# Autodesk Inventor assembly: Electrical Workbench
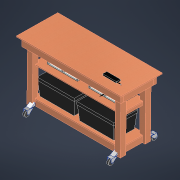
[picture p0: Inventor's stored thumbnail of the model, 180x180]
Saved by Autodesk Inventor 2022.3 (Build 263350000, 350)
## iProperties
Created: 2022-08-14
Part Number: Electrical Workbench
Document SubType Name: Assembly
Designer: hawle
Author: hawle
## Documents named in this file (25)
- G:\Robotics 2022 CAD Files\Workshop\Electrical Workbench.iam
- G:\Robotics 2022 CAD Files\Workshop\2x6x72 wood.ipt
- G:\Robotics 2022 CAD Files\Workshop\2x6x44 wood.ipt
- G:\Robotics 2022 CAD Files\Workshop\2x6x40 wood.ipt
- G:\Robotics 2022 CAD Files\Workshop\2x6x60 wood.ipt
- G:\Robotics 2022 CAD Files\Workshop\Workbench top.ipt
- G:\Robotics 2022 CAD Files\Workshop\workbench floor.ipt
- G:\Robotics 2022 CAD Files\Workshop\2x6x33 wood.ipt
- G:\Robotics 2022 CAD Files\Workshop\Workbench caster assembly.iam
- G:\Robotics 2022 CAD Files\Workshop\Power Strip.ipt
- G:\Robotics 2022 CAD Files\Game Pieces\First Tote.ipt
- G:\Robotics 2022 CAD Files\Workshop\Electrical Drawer.iam
- G:\Robotics 2022 CAD Files\Workshop\3x3x42 wood.ipt
- G:\Robotics 2022 CAD Files\Workshop\Electrical Workbench\AIP\FEA\e2dqfnm0w.fins
- G:\Robotics 2022 CAD Files\Workshop\Electrical Workbench\AIP\FEA\e2dqfnm0w.fsat
- G:\Robotics 2022 CAD Files\Workshop\Electrical Workbench\AIP\FEA\e2dqfnm0w.ftes
- G:\Robotics 2022 CAD Files\Workshop\Electrical Workbench\AIP\FEA\e2dqfnm0w.fwiz
- G:\Robotics 2022 CAD Files\Workshop\Electrical Workbench\AIP\FEA\e2dqfnm4g.fmsh
- G:\Robotics 2022 CAD Files\Workshop\Electrical Workbench\AIP\FEA\e2dqfnm5c.fres
- G:\Robotics 2022 CAD Files\Workshop\Electrical Workbench\AIP\FEA\e2kkncozk.fins
- G:\Robotics 2022 CAD Files\Workshop\Electrical Workbench\AIP\FEA\e2kkncozk.fsat
- G:\Robotics 2022 CAD Files\Workshop\Electrical Workbench\AIP\FEA\e2kkncozk.ftes
- G:\Robotics 2022 CAD Files\Workshop\Electrical Workbench\AIP\FEA\e2kkncozk.fwiz
- G:\Robotics 2022 CAD Files\Workshop\Electrical Workbench\AIP\FEA\e2kkncpeo.fmsh
- G:\Robotics 2022 CAD Files\Workshop\Electrical Workbench\AIP\FEA\e2kkncpep.fres
## Components (31 placed, 12 different names)
1. 2x6x72 wood:1 — Flush:18, Mate:27, Flush:70, Flush:96, Mate:96, Mate:97
2. 2x6x72 wood:2 — Mate:7, Flush:19, Flush:20, Mate:9, Flush:21, Mate:30, Mate:50, Mate:51, Flush:81, Mate:78, Mate:80, Flush:97
3. 2x6x44 wood:1 — Flush:18, Mate:7, Flush:19, Flush:20, Mate:35, Flush:82, Mate:79, Mate:84
4. 2x6x44 wood:2 — Mate:9, Flush:21, Mate:31, Mate:34, Mate:82, Mate:83, Flush:97
5. Workbench top:1 — Mate:27, Mate:29, Mate:32, Mate:33, Mate:64, Flush:71, Flush:81, Flush:82, Mate:86, Mate:87, Mate:88, Mate:89, Flush:96
6. 2x6x44 wood:3 — Mate:29, Mate:30, Mate:31, Flush:38, Flush:39, Mate:65
7. 2x6x33 wood:1 — Mate:33, Mate:35, Flush:38, Mate:51
8. 2x6x33 wood:2 — Mate:32, Mate:34, Flush:39, Mate:50
9. Power Strip:1 — Mate:64, Flush:70, Flush:71
10. Workbench caster assembly:1 [sub-assembly]
11. Workbench caster assembly:2 [sub-assembly] — Flush:69
12. Workbench caster assembly:3 [sub-assembly] — Flush:69
13. Workbench caster assembly:4 [sub-assembly]
14. First Tote:1 — Mate:63
15. 2x6x40 wood:1 — Flush:89, Flush:92, Mate:95
16. 2x6x40 wood:2 — Mate:59, Flush:61, Mate:60, Flush:88, Mate:98, Flush:101
17. 2x6x60 wood:1 — Mate:59, Flush:61, Flush:72, Flush:85, Flush:98
18. 2x6x60 wood:2 — Mate:60, Mate:62, Flush:88, Flush:89, Mate:94, Flush:95, Flush:99, Flush:100
19. workbench floor:1 — Mate:62, Mate:63, Mate:74, Flush:92, Flush:100, Flush:101
20. workbench floor:2 — Flush:72, Mate:65, Flush:74, Mate:66, Flush:75, Mate:69, Flush:79, Flush:80, Mate:76, Flush:86, Mate:77, Flush:87, Mate:99
21. Electrical Drawer:1 [sub-assembly] — Flush:74, Mate:66, Flush:75, Mate:67, Flush:76, Flush:83
22. Electrical Drawer:2 [sub-assembly] — Mate:67, Flush:76, Flush:83
23. Electrical Drawer:3 [sub-assembly] — Mate:69, Flush:78, Flush:79
24. Electrical Drawer:4 [sub-assembly] — Flush:78, Flush:80
25. First Tote:2 — Mate:74, Flush:85
26. 2x6x40 wood:3 — Mate:76, Flush:86, Mate:93
27. 2x6x40 wood:4 — Mate:77, Flush:87, Mate:92
28. 3x3x42 wood:1 — Mate:78, Mate:84, Mate:86, Mate:95
29. 3x3x42 wood:2 — Mate:79, Mate:87, Mate:92, Mate:94, Flush:95, Mate:96, Flush:99
30. 3x3x42 wood:3 — Mate:80, Mate:83, Mate:88, Mate:93, Flush:98
31. 3x3x42 wood:4 — Mate:82, Mate:89, Mate:97, Mate:98, Mate:99
## Relationships (77: Mate 43, Flush 34)
- Flush:18: 2x6x72 wood:1 ↔ 2x6x44 wood:1
- Mate:7: 2x6x72 wood:2 ↔ 2x6x44 wood:1
- Flush:19: 2x6x72 wood:2 ↔ 2x6x44 wood:1
- Flush:20: 2x6x72 wood:2 ↔ 2x6x44 wood:1
- Mate:9: 2x6x72 wood:2 ↔ 2x6x44 wood:2
- Flush:21: 2x6x72 wood:2 ↔ 2x6x44 wood:2
- Mate:27: 2x6x72 wood:1 ↔ Workbench top:1
- Mate:29: Workbench top:1 ↔ 2x6x44 wood:3
- Mate:30: 2x6x72 wood:2 ↔ 2x6x44 wood:3
- Mate:31 (838.2 mm): 2x6x44 wood:2 ↔ 2x6x44 wood:3
- Mate:32: Workbench top:1 ↔ 2x6x33 wood:2
- Mate:33: Workbench top:1 ↔ 2x6x33 wood:1
- Mate:34: 2x6x44 wood:2 ↔ 2x6x33 wood:2
- Mate:35: 2x6x44 wood:1 ↔ 2x6x33 wood:1
- Flush:38: 2x6x44 wood:3 ↔ 2x6x33 wood:1
- Flush:39: 2x6x44 wood:3 ↔ 2x6x33 wood:2
- Mate:50 (254 mm): 2x6x72 wood:2 ↔ 2x6x33 wood:2
- Mate:51 (254 mm): 2x6x72 wood:2 ↔ 2x6x33 wood:1
- Mate:59: 2x6x40 wood:2 ↔ 2x6x60 wood:1
- Flush:61: 2x6x40 wood:2 ↔ 2x6x60 wood:1
- Mate:60: 2x6x40 wood:2 ↔ 2x6x60 wood:2
- Mate:62: 2x6x60 wood:2 ↔ workbench floor:1
- Flush:69: Workbench caster assembly:2 ↔ Workbench caster assembly:3
- Mate:63: First Tote:1 ↔ workbench floor:1
- Mate:64: Workbench top:1 ↔ Power Strip:1
- Flush:70 (114.3 mm): 2x6x72 wood:1 ↔ Power Strip:1
- Flush:71 (247.65 mm): Workbench top:1 ↔ Power Strip:1
- Flush:72: 2x6x60 wood:1 ↔ workbench floor:2
- Mate:65 (254 mm): 2x6x44 wood:3 ↔ workbench floor:2
- Flush:74: workbench floor:2 ↔ Electrical Drawer:1
- Mate:66: workbench floor:2 ↔ Electrical Drawer:1
- Flush:75 (152.4 mm): workbench floor:2 ↔ Electrical Drawer:1
- Mate:67: Electrical Drawer:1 ↔ Electrical Drawer:2
- Flush:76: Electrical Drawer:1 ↔ Electrical Drawer:2
- [Mate]: Electrical Drawer:3 ↔ Electrical Drawer:4
- [Flush]: Electrical Drawer:3 ↔ Electrical Drawer:4
- Mate:69: workbench floor:2 ↔ Electrical Drawer:3
- Flush:78: Electrical Drawer:3 ↔ Electrical Drawer:4
- Flush:79: workbench floor:2 ↔ Electrical Drawer:3
- Flush:80 (152.4 mm): workbench floor:2 ↔ Electrical Drawer:4
- Flush:81 (50.8 mm): 2x6x72 wood:2 ↔ Workbench top:1
- Flush:82 (50.8 mm): 2x6x44 wood:1 ↔ Workbench top:1
- Flush:83: Electrical Drawer:1 ↔ Electrical Drawer:2
- Mate:74: workbench floor:1 ↔ First Tote:2
- Flush:85: 2x6x60 wood:1 ↔ First Tote:2
- Mate:76: workbench floor:2 ↔ 2x6x40 wood:3
- Flush:86: workbench floor:2 ↔ 2x6x40 wood:3
- Mate:77: workbench floor:2 ↔ 2x6x40 wood:4
- Flush:87: workbench floor:2 ↔ 2x6x40 wood:4
- Flush:88: 2x6x40 wood:2 ↔ 2x6x60 wood:2
- Flush:89: 2x6x40 wood:1 ↔ 2x6x60 wood:2
- Mate:78: 2x6x72 wood:2 ↔ 3x3x42 wood:1
- Mate:79: 2x6x44 wood:1 ↔ 3x3x42 wood:2
- Mate:80: 2x6x72 wood:2 ↔ 3x3x42 wood:3
- Mate:82: 2x6x44 wood:2 ↔ 3x3x42 wood:4
- Mate:83: 2x6x44 wood:2 ↔ 3x3x42 wood:3
- Mate:84: 2x6x44 wood:1 ↔ 3x3x42 wood:1
- Mate:86: Workbench top:1 ↔ 3x3x42 wood:1
- Mate:87: Workbench top:1 ↔ 3x3x42 wood:2
- Mate:88: Workbench top:1 ↔ 3x3x42 wood:3
- Mate:89: Workbench top:1 ↔ 3x3x42 wood:4
- Flush:92: 2x6x40 wood:1 ↔ workbench floor:1
- Mate:92: 2x6x40 wood:4 ↔ 3x3x42 wood:2
- Mate:93: 2x6x40 wood:3 ↔ 3x3x42 wood:3
- Mate:94: 2x6x60 wood:2 ↔ 3x3x42 wood:2
- Flush:95: 2x6x60 wood:2 ↔ 3x3x42 wood:2
- Mate:95: 2x6x40 wood:1 ↔ 3x3x42 wood:1
- Flush:96 (50.8 mm): 2x6x72 wood:1 ↔ Workbench top:1
- Mate:96: 2x6x72 wood:1 ↔ 3x3x42 wood:2
- Mate:97: 2x6x72 wood:1 ↔ 3x3x42 wood:4
- Flush:97: 2x6x72 wood:2 ↔ 2x6x44 wood:2
- Flush:98: 2x6x60 wood:1 ↔ 3x3x42 wood:3
- Flush:99: 2x6x60 wood:2 ↔ 3x3x42 wood:2
- Mate:98: 2x6x40 wood:2 ↔ 3x3x42 wood:4
- Flush:100: 2x6x60 wood:2 ↔ workbench floor:1
- Flush:101: 2x6x40 wood:2 ↔ workbench floor:1
- Mate:99: workbench floor:2 ↔ 3x3x42 wood:4
## Named parameters: sa_0 = 444822, d182_d180 = 0 mm, d183_d181 = 0 mm, sa_1 = 444822, sa_2 = 222411
note: some values were not read from the file. Shown as the stored number, unit unknown: "sa_0", "sa_1", "sa_2".
